# Autodesk Inventor assembly: GearBox_ProperConstraints
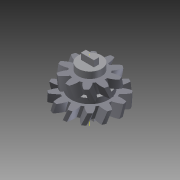
[picture p0: Inventor's stored thumbnail of the model, 180x180]
Saved by Autodesk Inventor 2012 (Build 160160000, 160)
## iProperties
Created: 2011-10-22
Part Number: GearBox_ProperConstraints
Document SubType Name: Assembly
Designer: KuttaA
Mass: 38.985 g
Surface Area: 178.451 cm^2
Volume: 22.0215 cm^3
Density: 1.77031 g/cm^3
Author: KuttaA
## Documents named in this file (7)
- C:\Users\akutta\Dropbox\Hexapod Research\Leg Design\Other Parts\Intermediary Gear Box\GearBox_ProperConstraints.iam
- C:\Users\akutta\Dropbox\Hexapod Research\Leg Design\Other Parts\Intermediary Gear Box\GearboxWallOutput.ipt
- C:\Users\akutta\Dropbox\Hexapod Research\Leg Design\Other Parts\Intermediary Gear Box\LargeSmallGearAxis.ipt
- C:\Users\akutta\Dropbox\Hexapod Research\Leg Design\Other Parts\Intermediary Gear Box\DerivedPartsFromAssemblies\LargeGearInput.ipt
- C:\Users\akutta\Dropbox\Hexapod Research\Leg Design\Other Parts\Intermediary Gear Box\DerivedPartsFromAssemblies\TransferGear.ipt
- C:\Users\akutta\Dropbox\Hexapod Research\Leg Design\Other Parts\Intermediary Gear Box\GearBoxTop.ipt
- C:\Users\akutta\Dropbox\Hexapod Research\Leg Design\Other Parts\Intermediary Gear Box\SmallGearOutput.ipt
## Components (6 placed, 6 different names)
1. GearboxWallOutput:1 — Mate:1, Mate:6, Mate:7, Mate:8, Mate:11, Mate:12, Mate:16, Mate:17, Mate:18, Mate:19, Mate:20
2. LargeSmallGearAxis:1 — Mate:6, Mate:7, Mate:8, Mate:9, Mate:21
3. LargeGearInput:1 — Mate:11, Mate:12, Rotation:1
4. TransferGear:1 — Mate:9, Rotation:1, Mate:21
5. GearBoxTop:1 — Mate:16, Mate:17, Mate:18
6. Spur Gear1:1 — Mate:19, Mate:20
## Relationships (14: Mate 13, RelateRotation 1)
- Mate:1: GearboxWallOutput:1
- Mate:6 (3 mm): GearboxWallOutput:1 ↔ LargeSmallGearAxis:1
- Mate:7 (0.3 mm): GearboxWallOutput:1 ↔ LargeSmallGearAxis:1
- Mate:8 (0.3 mm): GearboxWallOutput:1 ↔ LargeSmallGearAxis:1
- Mate:9: LargeSmallGearAxis:1 ↔ TransferGear:1
- Mate:11: GearboxWallOutput:1 ↔ LargeGearInput:1
- Mate:12 (0.3 mm): GearboxWallOutput:1 ↔ LargeGearInput:1
- Rotation:1 [RelateRotation] (0.7692 ul): LargeGearInput:1 ↔ TransferGear:1
- Mate:16: GearboxWallOutput:1 ↔ GearBoxTop:1
- Mate:17 (0.3 mm): GearboxWallOutput:1 ↔ GearBoxTop:1
- Mate:18 (0.3 mm): GearboxWallOutput:1 ↔ GearBoxTop:1
- Mate:19 (0.3 mm): GearboxWallOutput:1 ↔ Spur Gear1:1
- Mate:20: GearboxWallOutput:1 ↔ Spur Gear1:1
- Mate:21 (0.3 mm): LargeSmallGearAxis:1 ↔ TransferGear:1
